# Autodesk Inventor assembly: Assy_fork_connection
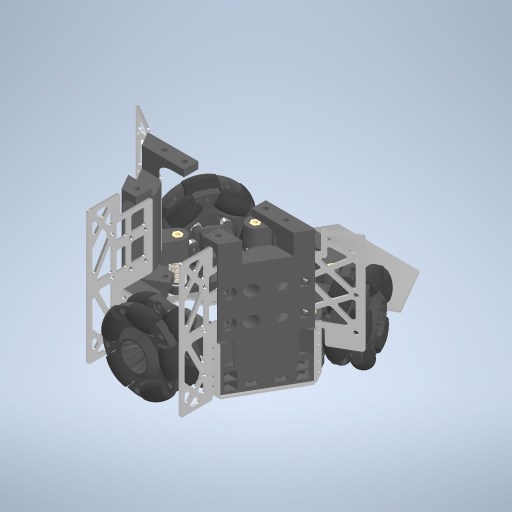
[picture p0: Inventor's stored thumbnail of the model, 512x512]
Saved by Autodesk Inventor 2024.1 (Build 281209000, 209)
## iProperties
Created: 2025-03-04
Part Number: Assy_fork_connection
Document SubType Name: Assembly
Designer: hibik
Author: hibik
## Documents named in this file (4)
- C:\Users\hibik\Documents\Robomech\RESCUE\ORCA\hard\Assy_fork_connection.iam
- C:\Users\hibik\Documents\Robomech\RESCUE\ORCA\hard\Assy_foot.iam
- C:\Users\hibik\Documents\Robomech\RESCUE\ORCA\hard\flame_base\base2fork_connecter_front.ipt
- C:\Users\hibik\Documents\Robomech\RESCUE\ORCA\hard\flame_base\base2fork_connecter_back.ipt
## Components (5 placed, 3 different names)
1. Assy_foot:1 [sub-assembly] — 挿入:1, 挿入:2, 挿入:3, 挿入:4, 挿入:8, 挿入:9, 挿入:10, 挿入:11
2. base2fork_connecter_back:1 — 挿入:1, 挿入:2
3. base2fork_connecter_front:1 — 挿入:3, 挿入:4
4. base2fork_connecter_front:2 — 挿入:10, 挿入:11
5. base2fork_connecter_back:2 — 挿入:8, 挿入:9
## Relationships (8: Insert 8)
- 挿入:1 [Insert]: Assy_foot:1 ↔ base2fork_connecter_back:1
- 挿入:2 [Insert]: Assy_foot:1 ↔ base2fork_connecter_back:1
- 挿入:3 [Insert]: Assy_foot:1 ↔ base2fork_connecter_front:1
- 挿入:4 [Insert]: Assy_foot:1 ↔ base2fork_connecter_front:1
- 挿入:8 [Insert]: Assy_foot:1 ↔ base2fork_connecter_back:2
- 挿入:9 [Insert]: Assy_foot:1 ↔ base2fork_connecter_back:2
- 挿入:10 [Insert]: Assy_foot:1 ↔ base2fork_connecter_front:2
- 挿入:11 [Insert]: Assy_foot:1 ↔ base2fork_connecter_front:2
